# Autodesk Inventor assembly: SwerveDriveMotorASM
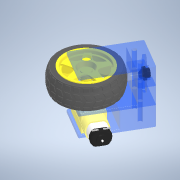
[picture p0: Inventor's stored thumbnail of the model, 180x180]
Saved by Autodesk Inventor 2022.3 (Build 263350000, 350)
## iProperties
Created: 2022-06-17
Part Number: SwerveDriveMotorASM
Document SubType Name: Assembly
Designer: Robert Nies
Author: Robert Nies
## Documents named in this file (5)
- C:\Users\rober\PycharmProjects\SwervoDrive\CAD\SwerveDriveMotorASM.iam
- C:\Users\rober\PycharmProjects\SwervoDrive\CAD\SwerveDriveBracketASM.iam
- C:\Users\rober\PycharmProjects\SwervoDrive\CAD\CAD_Lib\Servo\attachmentStraight.ipt
- C:\Users\rober\PycharmProjects\SwervoDrive\CAD\CAD_Lib\drive_motor.ipt
- C:\Users\rober\PycharmProjects\SwervoDrive\CAD\CAD_Lib\wheel.ipt
## Components (4 placed, 4 different names)
1. SwerveDriveBracketASM:1 [sub-assembly] — Rotational:1, Rotational:2, Rotational:3
2. attachmentStraight:1 — Rotational:1
3. drive_motor:1 — Mate:1, Mate:2, Mate:3, Rotational:2, Rotational:3
4. wheel:1 — Mate:1, Mate:2, Mate:3
## Relationships (6: RevoluteJoint 3, Mate 3)
- Rotational:1 [RevoluteJoint]: SwerveDriveBracketASM:1 ↔ attachmentStraight:1
- Mate:1 (1.5875 mm): drive_motor:1 ↔ wheel:1
- Mate:2: drive_motor:1 ↔ wheel:1
- Mate:3: drive_motor:1 ↔ wheel:1
- Rotational:2 [RevoluteJoint]: SwerveDriveBracketASM:1 ↔ drive_motor:1
- Rotational:3 [RevoluteJoint]: SwerveDriveBracketASM:1 ↔ drive_motor:1
